# Autodesk Inventor assembly: Assembly_Cube_Sampleholder
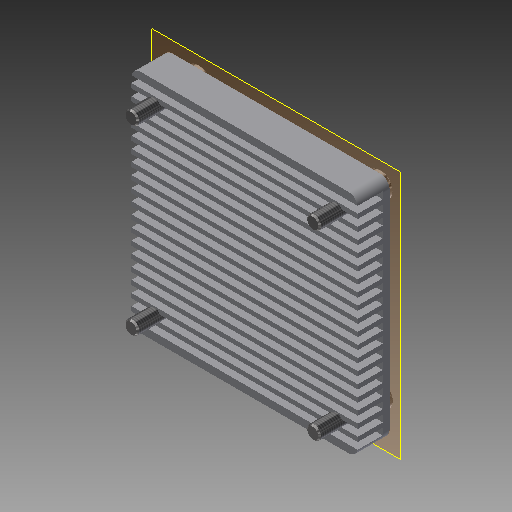
[picture p0: Inventor's stored thumbnail of the model, 512x512]
Saved by Autodesk Inventor 2019 (Build 230136000, 136)
## iProperties
Created: 2020-12-04
Part Number: Assembly_Cube_Sampleholder
Document SubType Name: Assembly
Designer: UC2
Author: UC2
## Documents named in this file (3)
- C:\Users\marsikovabarbora\Dropbox\UC2\02_CAD\INVENTOR\uc2_v3\Assembly_Cube_Sampleholder.iam
- C:\Users\marsikovabarbora\Dropbox\UC2\02_CAD\INVENTOR\uc2_v3\30_Cube_sampleholder.ipt
- C:\Users\marsikovabarbora\Documents\Inventor\Content Center Files\R2019\en-US\DIN 912\DIN 912 - M3 x 0,5 x 12 x 10,75.ipt
## Components (5 placed, 2 different names)
1. 30_Cube_sampleholder:1 — Passend:1, Passend:2, Passend:3, Passend:4, Passend:5
2. DIN 912 - replaced by DIN EN ISO 4762 M3 x 12:1 — Passend:1, Fluchtend:1, Fluchtend:2, Fluchtend:3, Passend:5
3. DIN 912 - replaced by DIN EN ISO 4762 M3 x 12:2 — Passend:2, Fluchtend:1
4. DIN 912 - replaced by DIN EN ISO 4762 M3 x 12:3 — Passend:3, Fluchtend:2
5. DIN 912 - replaced by DIN EN ISO 4762 M3 x 12:4 — Passend:4, Fluchtend:3
## Relationships (8: Mate 5, Flush 3)
- Passend:1 [Mate]: 30_Cube_sampleholder:1 ↔ DIN 912 - replaced by DIN EN ISO 4762 M3 x 12:1
- Passend:2 [Mate]: 30_Cube_sampleholder:1 ↔ DIN 912 - replaced by DIN EN ISO 4762 M3 x 12:2
- Passend:3 [Mate]: 30_Cube_sampleholder:1 ↔ DIN 912 - replaced by DIN EN ISO 4762 M3 x 12:3
- Passend:4 [Mate]: 30_Cube_sampleholder:1 ↔ DIN 912 - replaced by DIN EN ISO 4762 M3 x 12:4
- Fluchtend:1 [Flush]: DIN 912 - replaced by DIN EN ISO 4762 M3 x 12:1 ↔ DIN 912 - replaced by DIN EN ISO 4762 M3 x 12:2
- Fluchtend:2 [Flush]: DIN 912 - replaced by DIN EN ISO 4762 M3 x 12:1 ↔ DIN 912 - replaced by DIN EN ISO 4762 M3 x 12:3
- Fluchtend:3 [Flush]: DIN 912 - replaced by DIN EN ISO 4762 M3 x 12:1 ↔ DIN 912 - replaced by DIN EN ISO 4762 M3 x 12:4
- Passend:5 [Mate]: 30_Cube_sampleholder:1 ↔ DIN 912 - replaced by DIN EN ISO 4762 M3 x 12:1
